# Autodesk Inventor assembly: Assembly2
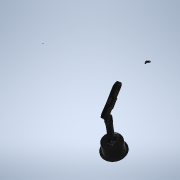
[picture p0: Inventor's stored thumbnail of the model, 180x180]
Saved by Autodesk Inventor 2022 (Build 260153000, 153)
## iProperties
Created: 2021-06-19
Part Number: Assembly2
Document SubType Name: Assembly
Designer: Nay
Author: Nay
## Documents named in this file (7)
- C:\Users\Nay\Documents\Assembly2.iam
- C:\Users\Nay\Documents\الذراع\Imported Components\Arm 01\Arm 01.ipt
- C:\Users\Nay\Documents\الذراع\Imported Components\Base\Base.ipt
- C:\Users\Nay\Documents\Inventor\Content Center Files\R2022\الذراع\Imported Components\Waist\Waist.ipt
- C:\Users\Nay\Documents\Inventor\Content Center Files\R2022\الذراع\Imported Components\Cube.002\Cube.002.ipt
- C:\Users\Nay\Documents\Inventor\Content Center Files\R2022\الذراع\Imported Components\Gripper\Gripper.ipt
- C:\Users\Nay\Documents\Inventor\Content Center Files\R2022\الذراع\Imported Components\Arm 02\Arm 02.ipt
## Components (6 placed, 6 different names)
1. Arm 01:1 — Rotational:2, Rotational:3
2. Base:1 — Rotational:1
3. Waist:1 — Rotational:1, Rotational:2
4. Cube.002:1
5. Gripper:1
6. Arm 02:1 — Rotational:3
## Relationships (3: RevoluteJoint 3)
- Rotational:1 [RevoluteJoint]: Base:1 ↔ Waist:1
- Rotational:2 [RevoluteJoint]: Arm 01:1 ↔ Waist:1
- Rotational:3 [RevoluteJoint]: Arm 01:1 ↔ Arm 02:1
